# Autodesk Inventor assembly: Montagem_MANIPULADOR
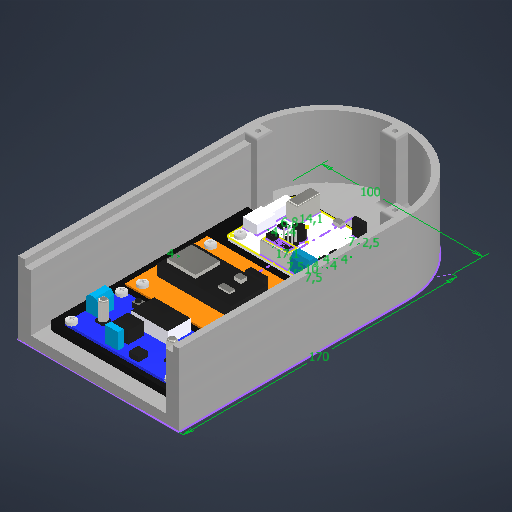
[picture p0: Inventor's stored thumbnail of the model, 512x512]
Saved by Autodesk Inventor 2027.1 (Build 311270010, 270A)
## iProperties
Created: 2026-08-16
Part Number: Montagem_MANIPULADOR
Document SubType Name: Assembly
Designer: Evellyn
Author: Evellyn
## Documents named in this file (3)
- C:\Users\Evellyn\Desktop\New-Robotic-Arm\mecanica\partes_ipt\Montagem_MANIPULADOR.iam
- C:\Users\Evellyn\Desktop\New-Robotic-Arm\mecanica\partes_ipt\BASE_MANIPULADOR.ipt
- C:\Users\Evellyn\Desktop\New-Robotic-Arm\mecanica\partes_ipt\MONTAGEM_BASE_ELETRONICA.iam
## Components (2 placed, 2 different names)
1. BASE_MANIPULADOR:1 — Coincidente:1, Coincidente:2, Coincidente:3, Coincidente:4, Coincidente:5, Coincidente:6, Coincidente:7
2. MONTAGEM_BASE_ELETRONICA:1 [sub-assembly] — Coincidente:4, Coincidente:5, Coincidente:6, Coincidente:7
## Relationships (7: Mate 7)
- Coincidente:1 [Mate]: BASE_MANIPULADOR:1
- Coincidente:2 [Mate]: BASE_MANIPULADOR:1
- Coincidente:3 [Mate]: BASE_MANIPULADOR:1
- Coincidente:4 [Mate]: BASE_MANIPULADOR:1 ↔ MONTAGEM_BASE_ELETRONICA:1
- Coincidente:5 [Mate]: BASE_MANIPULADOR:1 ↔ MONTAGEM_BASE_ELETRONICA:1
- Coincidente:6 [Mate]: BASE_MANIPULADOR:1 ↔ MONTAGEM_BASE_ELETRONICA:1
- Coincidente:7 [Mate]: BASE_MANIPULADOR:1 ↔ MONTAGEM_BASE_ELETRONICA:1
